# Autodesk Inventor assembly: sestava estonsko
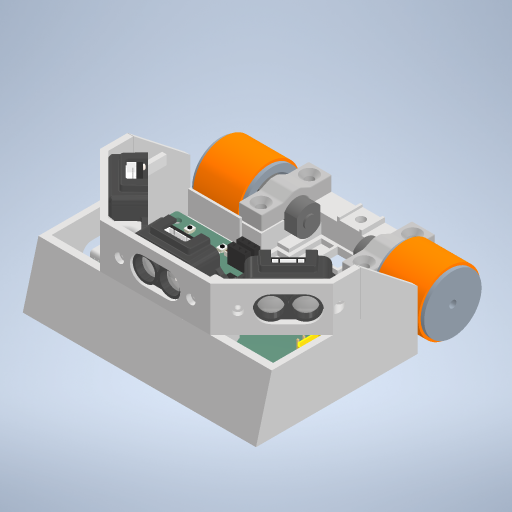
[picture p0: Inventor's stored thumbnail of the model, 512x512]
Saved by Autodesk Inventor 2024 (Build 280153000, 153)
## iProperties
Created: 2023-10-31
Part Number: sestava estonsko
Document SubType Name: Assembly
Designer: Simak
Author: Simak
## Documents named in this file (7)
- C:\Users\Simak\OneDrive\Dokumenty\GitHub\RoboCop\- 3D -\wip\sestava estonsko.iam
- C:\Users\Simak\OneDrive\Dokumenty\GitHub\RoboCop\- 3D -\el._parts\sumec\sumec.ipt
- C:\Users\Simak\OneDrive\Dokumenty\GitHub\RoboCop\- 3D -\wip\tělo estonsko.ipt
- C:\Users\Simak\OneDrive\Dokumenty\GitHub\RoboCop\- 3D -\wip\Sestava TF-Luna a držáku.iam
- C:\Users\Simak\OneDrive\Dokumenty\GitHub\RoboCop\- 3D -\el._parts\GA12-N20_Motor.ipt
- C:\Users\Simak\OneDrive\Dokumenty\GitHub\RoboCop\- 3D -\mech._parts\wheel+silicon.ipt
- C:\Users\Simak\OneDrive\Dokumenty\GitHub\RoboCop\- 3D -\mech._parts\motor_C_clamp.ipt
## Components (9 placed, 6 different names)
1. tělo estonsko:1 — Tuhé:1, Vložit:3, Proti sobě:2, Proti sobě:3, Vložit:4, Vložit:5, Vložit:6, Proti sobě:4, Proti sobě:5, Proti sobě:7, Proti sobě:9, Proti sobě:10, Vložit:7, Vložit:8
2. sumec:1 — Proti sobě:3, Vložit:4, Vložit:5
3. Sestava TF-Luna a držáku:1 [sub-assembly] — Tuhé:1
4. GA12-N20_Motor:1 — Vložit:3, Proti sobě:2, Proti sobě:6, Proti sobě:11
5. GA12-N20_Motor:2 — Vložit:6, Proti sobě:4, Proti sobě:8, Proti sobě:12
6. wheel+silicon:1 — Proti sobě:5, Proti sobě:6
7. wheel+silicon:2 — Proti sobě:7, Proti sobě:8
8. motor_C_clamp:1 — Proti sobě:9, Vložit:7, Proti sobě:11
9. motor_C_clamp:2 — Proti sobě:10, Vložit:8, Proti sobě:12
## Relationships (18: Mate 11, Insert 6, WeldJoint 1)
- Tuhé:1 [WeldJoint]: tělo estonsko:1 ↔ Sestava TF-Luna a držáku:1
- Vložit:3 [Insert]: tělo estonsko:1 ↔ GA12-N20_Motor:1
- Proti sobě:2 [Mate]: tělo estonsko:1 ↔ GA12-N20_Motor:1
- Proti sobě:3 [Mate]: tělo estonsko:1 ↔ sumec:1
- Vložit:4 [Insert]: tělo estonsko:1 ↔ sumec:1
- Vložit:5 [Insert]: tělo estonsko:1 ↔ sumec:1
- Vložit:6 [Insert]: tělo estonsko:1 ↔ GA12-N20_Motor:2
- Proti sobě:4 [Mate]: tělo estonsko:1 ↔ GA12-N20_Motor:2
- Proti sobě:5 [Mate] (0.5 mm): tělo estonsko:1 ↔ wheel+silicon:1
- Proti sobě:6 [Mate]: GA12-N20_Motor:1 ↔ wheel+silicon:1
- Proti sobě:7 [Mate] (0.5 mm): tělo estonsko:1 ↔ wheel+silicon:2
- Proti sobě:8 [Mate]: GA12-N20_Motor:2 ↔ wheel+silicon:2
- Proti sobě:9 [Mate]: tělo estonsko:1 ↔ motor_C_clamp:1
- Proti sobě:10 [Mate]: tělo estonsko:1 ↔ motor_C_clamp:2
- Vložit:7 [Insert]: tělo estonsko:1 ↔ motor_C_clamp:1
- Proti sobě:11 [Mate]: GA12-N20_Motor:1 ↔ motor_C_clamp:1
- Vložit:8 [Insert]: tělo estonsko:1 ↔ motor_C_clamp:2
- Proti sobě:12 [Mate]: GA12-N20_Motor:2 ↔ motor_C_clamp:2
